# Autodesk Inventor assembly: ASY MSC 900.2 support
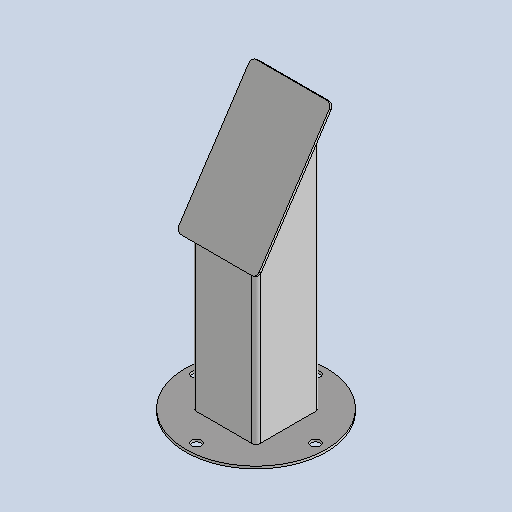
[picture p0: Inventor's stored thumbnail of the model, 512x512]
Saved by Autodesk Inventor 2025 (Build 290162010, 162A)
## iProperties
Created: 2024-08-15
Part Number: ASY MSC 900.2 support
Document SubType Name: Assembly
Designer: admin
Stock Number: ASY МОО 900.2 опора
Author: admin
Revision Number: 8
## Documents named in this file (4)
- C:\Users\admin\YandexDisk-badmisterfox\домашниий пк\Inventor\Manturovo\Manturovo_Se-clar\ASY MSC 900.2 support.iam
- C:\Users\admin\YandexDisk-badmisterfox\домашниий пк\Inventor\Manturovo\Manturovo_Se-clar\MSC 903 base tube.ipt
- C:\Users\admin\YandexDisk-badmisterfox\домашниий пк\Inventor\Manturovo\Manturovo_Se-clar\MSC 904 flange base tube.ipt
- C:\Users\admin\YandexDisk-badmisterfox\домашниий пк\Inventor\Manturovo\Manturovo_Se-clar\MSC 905 flange base tube support.ipt
## Components (3 placed, 3 different names)
1. MSC 903 base tube.ipt:1
2. MSC 904 flange base tube.ipt:1 — Mate:1, Mate:2, Mate:3, Mate:4
3. MSC 905 flange base tube support.ipt:1
## Relationships (6: Mate 4, WeldJoint 2)
- [WeldJoint]: MSC 903 base tube.ipt:1 ↔ MSC 904 flange base tube.ipt:1
- [WeldJoint]: MSC 903 base tube.ipt:1 ↔ MSC 905 flange base tube support.ipt:1
- Mate:1: MSC 904 flange base tube.ipt:1
- Mate:2: MSC 904 flange base tube.ipt:1
- Mate:3: MSC 904 flange base tube.ipt:1
- Mate:4: MSC 904 flange base tube.ipt:1
